# Autodesk Inventor assembly: BoronProbePipe
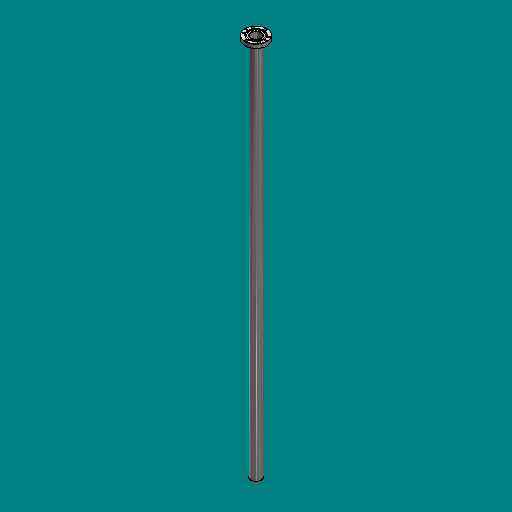
[picture p0: Inventor's stored thumbnail of the model, 512x512]
Saved by Autodesk Inventor 2025 (Build 290162000, 162)
## iProperties
Created: 2024-05-30
Part Number: BoronProbePipe
Document SubType Name: Assembly
Designer: kuzmin
Author: kuzmin
## Documents named in this file (3)
- C:\Users\queez\Dropbox\Drawings\PIHTI\BoronProbe\BoronProbePipe.iam
- C:\Users\queez\Dropbox\Drawings\PIHTI\PALP\Prototype-PALP-CF70-34-hole-flange.ipt
- C:\Users\queez\Dropbox\Drawings\PIHTI\BoronProbe\BoronProbePipeLong.ipt
## Components (2 placed, 2 different names)
1. BoronProbePipeLong:1
2. Prototype-PALP-CF70-34-hole-flange:1
## Relationships (1: WeldJoint 1)
- [WeldJoint]: BoronProbePipeLong:1 ↔ Prototype-PALP-CF70-34-hole-flange:1
